# Autodesk Inventor assembly: A2017_T3_01
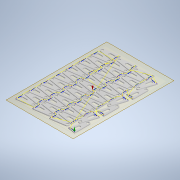
[picture p0: Inventor's stored thumbnail of the model, 180x180]
Saved by Autodesk Inventor 2022 (Build 260153000, 153)
## iProperties
Created: 2022-09-28
Part Number: A2017_T3_01
Document SubType Name: Assembly
Designer: Masato
Author: Masato
## Documents named in this file (3)
- C:\Users\6343y\ドキュメント\Inventor\SUSTAINA-OP\Cam\A2017_T3\A2017_T3_01.iam
- C:\Users\6343y\ドキュメント\Inventor\SUSTAINA-OP\Cam\DisposableBoard.ipt
- C:\Users\6343y\ドキュメント\Inventor\SUSTAINA-OP\LowerBody\Leg_joint\Leg_joint_slider_frame.ipt
## Components (49 placed, 2 different names)
1. DisposableBoard:1 — フラッシュ:1, フラッシュ:2, フラッシュ:3, フラッシュ:4, フラッシュ:5, フラッシュ:6, 正接:1, フラッシュ:7, 正接:2, メイト:5
2. Leg_joint_slider_frame:2 — メイト:1, メイト:3, 正接:1
3. Leg_joint_slider_frame:1 — メイト:2, メイト:3, フラッシュ:5, フラッシュ:6
4. Leg_joint_slider_frame:3
5. Leg_joint_slider_frame:4
6. Leg_joint_slider_frame:5
7. Leg_joint_slider_frame:6
8. Leg_joint_slider_frame:7
9. Leg_joint_slider_frame:8
10. Leg_joint_slider_frame:9
11. Leg_joint_slider_frame:10
12. Leg_joint_slider_frame:11 — メイト:7
13. Leg_joint_slider_frame:12
14. Leg_joint_slider_frame:13
15. Leg_joint_slider_frame:14
16. Leg_joint_slider_frame:15
17. Leg_joint_slider_frame:16
18. Leg_joint_slider_frame:17
19. Leg_joint_slider_frame:18
20. Leg_joint_slider_frame:19
21. Leg_joint_slider_frame:20
22. Leg_joint_slider_frame:21
23. Leg_joint_slider_frame:22
24. Leg_joint_slider_frame:23
25. Leg_joint_slider_frame:24
26. Leg_joint_slider_frame:25
27. Leg_joint_slider_frame:26
28. Leg_joint_slider_frame:27
29. Leg_joint_slider_frame:28
30. Leg_joint_slider_frame:29
31. Leg_joint_slider_frame:30
32. Leg_joint_slider_frame:31
33. Leg_joint_slider_frame:32
34. Leg_joint_slider_frame:33
35. Leg_joint_slider_frame:34
36. Leg_joint_slider_frame:35
37. Leg_joint_slider_frame:36
38. Leg_joint_slider_frame:37
39. Leg_joint_slider_frame:38
40. Leg_joint_slider_frame:39
41. Leg_joint_slider_frame:40
42. Leg_joint_slider_frame:41
43. Leg_joint_slider_frame:42
44. Leg_joint_slider_frame:43 — メイト:4, フラッシュ:7, 正接:2, メイト:6
45. Leg_joint_slider_frame:44 — メイト:5, メイト:6, メイト:7
46. Leg_joint_slider_frame:45
47. Leg_joint_slider_frame:46
48. Leg_joint_slider_frame:47
49. Leg_joint_slider_frame:48
## Component patterns: (21 elements, first: Leg_joint_slider_frame:2 + Leg_joint_slider_frame:1), (3 elements, first: Leg_joint_slider_frame:43 + Leg_joint_slider_frame:44)
## Relationships (16: Flush 7, Mate 7, Tangent 2)
- フラッシュ:1 [Flush]: DisposableBoard:1
- フラッシュ:2 [Flush]: DisposableBoard:1
- フラッシュ:3 [Flush]: DisposableBoard:1
- フラッシュ:4 [Flush]: DisposableBoard:1
- メイト:1 [Mate]: Leg_joint_slider_frame:2
- メイト:2 [Mate]: Leg_joint_slider_frame:1
- メイト:3 [Mate] (2.1 mm): Leg_joint_slider_frame:2 ↔ Leg_joint_slider_frame:1
- フラッシュ:5 [Flush] (2.1 mm): DisposableBoard:1 ↔ Leg_joint_slider_frame:1
- フラッシュ:6 [Flush] (2.1 mm): DisposableBoard:1 ↔ Leg_joint_slider_frame:1
- 正接:1 [Tangent] (2.1 mm): DisposableBoard:1 ↔ Leg_joint_slider_frame:2
- メイト:4 [Mate]: Leg_joint_slider_frame:43
- フラッシュ:7 [Flush] (2.1 mm): DisposableBoard:1 ↔ Leg_joint_slider_frame:43
- 正接:2 [Tangent] (3.5 mm): DisposableBoard:1 ↔ Leg_joint_slider_frame:43
- メイト:5 [Mate]: DisposableBoard:1 ↔ Leg_joint_slider_frame:44
- メイト:6 [Mate] (2.1 mm): Leg_joint_slider_frame:43 ↔ Leg_joint_slider_frame:44
- メイト:7 [Mate] (2.1 mm): Leg_joint_slider_frame:11 ↔ Leg_joint_slider_frame:44
